# Autodesk Inventor assembly: realsense_backplate_bg
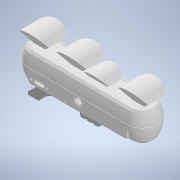
[picture p0: Inventor's stored thumbnail of the model, 180x180]
Saved by Autodesk Inventor 2021.3 (Build 253353010, 353A)
## iProperties
Created: 2021-08-11
Part Number: realsense_backplate_bg
Document SubType Name: Assembly
Designer: Markus
Author: Markus
## Documents named in this file (4)
- C:\Users\Markus\Documents\Inventor\Realsense\realsense_backplate_bg.iam
- C:\Users\Markus\Documents\Inventor\Realsense\realsense\Intel_RealSense_D455_CAD_external_v2.iam
- C:\Users\Markus\Documents\Inventor\Realsense\BackPlate.ipt
- C:\Users\Markus\Documents\Inventor\Realsense\Protector.ipt
## Components (3 placed, 3 different names)
1. Intel_RealSense_D455_CAD_external_v2:1 [sub-assembly] — Fluchtend:1
2. BackPlate:1 — Fluchtend:1, Fluchtend:2
3. Protector:1 — Fluchtend:2
## Relationships (2: Flush 2)
- Fluchtend:1 [Flush]: Intel_RealSense_D455_CAD_external_v2:1 ↔ BackPlate:1
- Fluchtend:2 [Flush]: BackPlate:1 ↔ Protector:1
